# Autodesk Inventor assembly: SCHUNK- 1321170 Co-act EGP-C 40-N-N-KTOE, 0
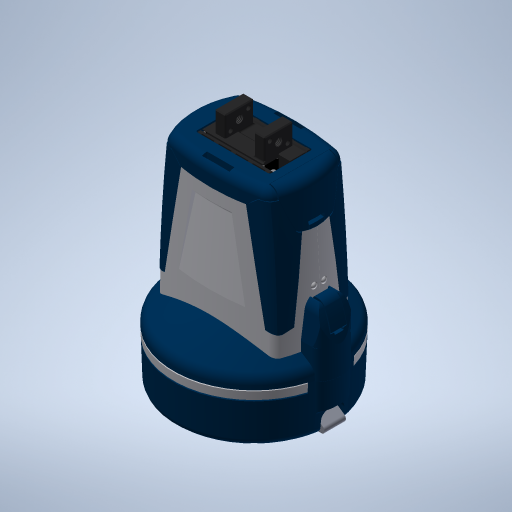
[picture p0: Inventor's stored thumbnail of the model, 512x512]
Saved by Autodesk Inventor 2023 (Build 270158000, 158)
## iProperties
Created: 2022-08-29
Part Number: SCHUNK- 1321170 Co-act EGP-C 40-N-N-KTOE, 0
Catalog Web Link: www.cadenas.de
Description: Co-act EGP-C-Collaborating gripper for small components
Vendor: SCHUNK
Document SubType Name: Assembly
Designer: psAdmin
Manufacturer: SCHUNK
Mass: 620 g
Surface Area: 1018.14 cm^2
Volume: 436.323 cm^3
Density: 1.42097 g/cm^3
Category: PARTsolutions
Company: SCHUNK
PSOL_IDENT_0: {$CADENAS_DATA/23d-libs/schunk/greifsysteme/greifmodule/co_act/co_act_egp_c/co_act_egp_c_asm_at.prj}
PSOL_IDENT_1: ,248 {VTYP=3D},{STYP=ASSTAB},{NB=SCHUNK- 1321170 Co-act EGP-C 40-N-N-KTOE, 0},{LINA=SCHUNK-1321170 C
PSOL_IDENT_2: o-act EGP-C 40-N-N-KTOE},{NN=Co-act EGP-C},{DATE=01.06.2022 15:24:31},{GEOMDATE=27.04.2022 08:42:34}
PSOL_IDENT_3: ,{VERSION=},{LINEID=20},{WBVAR=HUB},{WBNUMERIC=HUB}  {NB=SCHUNK- 1321170 Co-act EGP-C 40-N-N-KTOE, 0
PSOL_IDENT_4: },{LINA=SCHUNK-1321170 Co-act EGP-C 40-N-N-KTOE},{KT=DUMMY},{IDNR=1321170},{TYP=Co-act EGP-C 40-N-N-
PSOL_IDENT_5: KTOE},{ONLINE=Zur Produktseite},{INFOXX=https://schunk.com/gb_en/gripping-systems/product/63294-0},{
PSOL_IDENT_6: HUB=0},{CALC=../../../../produktbilder/icons/im0023672.png},{EPLAN=../../../../produktbilder/icons/i
PSOL_IDENT_7: m0021678.png},{HUBMAX=6.000},{PARTSERVER=1.000},{TYPBG=2.000},{TYP1=1.000},{TYPFLA=2.000},{WFLA=30.0
PSOL_IDENT_8: 00},{TYPEGP=EGP 40-N-N-B},{ROBOTER=KUKA LBR iiwa 7/14},{FLANSCH=Medien-Flansch Touch elektrisch},{LE
PSOL_IDENT_9: D=integriert},{FARBEN=Grün, Gelb, Rot},{SENSOREN=Ja, 2-fach induktiv},{HUBBACKE=6},{GREIFKRAFT=35/14
PSOL_IDENT_10: 0},{KRAFTPROBACKE=17.5/70},{WKSTGEWICHT=0.700},{FINGERLAENGE=50},{MASSEFINGER=0.080},{WIEDERHOLGENAU
PSOL_IDENT_11: I=0.020},{SCHLIESSOEFFNUN=0.2/0.2},{EIGENMASSE=0.620},{UMGEBUNGSTEMPER=5/55},{SCHUTZART=30},{KABELST
PSOL_IDENT_12: ECKEREND=M12},{KABELLAENGE=70},{NENNSPANN=24},{NENNSTROM=0.200},{MAXSTROM=2.000},{REGLERELEKTRONI=in
PSOL_IDENT_13: tegriert},{KOMMUNIKATIONSS=Digitale I/O},{ANZDIGITALEIO=4/2},{HOEHE=118.000},{HEGP=88.500},{CALCXX=h
PSOL_IDENT_14: ttps://schunk.com/de_de/services/digitale-services/berechnungs-und-auslegungstool-greifen/},{CALCXXX=
PSOL_IDENT_15: https://schunk.com/de_de/services/digitale-services/berechnungs-und-auslegungstool-greifen/},{EPLANX
PSOL_IDENT_16: X=https://eplandata.de/portal/portal.php?action=part-viewc&edpp=1.0&ev=1.9.11&lang=de_DE&clang=de_DE
PSOL_IDENT_17: &mf=SNK&lastmpg=.&mcat=_eplan&tab=c&mcatsel=SNK},{EPLANXXX=https://eplandata.de/portal/portal.php?ac
PSOL_IDENT_18: tion=part-viewc&edpp=1.0&ev=1.9.11&lang=de_DE&clang=de_DE&mf=SNK&lastmpg=.&mcat=_eplan&tab=c&mcatsel=
PSOL_IDENT_19: SNK},{CNSCTN=84798997},{EDZ=snk.1321170},{EPIMID=63294},{PPATH=co_act_egp_c_asmsbl.prj}
NB: SCHUNK- 1321170 Co-act EGP-C 40-N-N-KTOE, 0
NN: Co-act EGP-C
NT: Collaborating gripper for small components
NBSYN: SCHUNK- $IDNR. $TYP., $HUB.
LINA: SCHUNK-1321170 Co-act EGP-C 40-N-N-KTOE
CATALOG: SCHUNK
IDNR: 1321170
TYP: Co-act EGP-C 40-N-N-KTOE
ONLINE: To the product page
HUB: 0
CALC: ../../../../produktbilder/icons/im0023672.png
EPLAN: ../../../../produktbilder/icons/im0021678.png
ROBOTER: KUKA LBR iiwa 7/14
FLANSCH: Media flange touch electric
LED: integrated
FARBEN: green, yellow, red
SENSOREN: yes, inductive in two directions
HUBBACKE: 6
GREIFKRAFT: 35/140
KRAFTPROBACKE: 17.5/70
WKSTGEWICHT: 0.7
FINGERLAENGE: 50
MASSEFINGER: 0.08
WIEDERHOLGENAUI: 0.02
SCHLIESSOEFFNUN: 0.2/0.2
EIGENMASSE: 0.62
UMGEBUNGSTEMPER: 5/55
SCHUTZART: 30
KABELSTECKEREND: M12
KABELLAENGE: 70
NENNSPANN: 24
NENNSTROM: 0.2
MAXSTROM: 2
REGLERELEKTRONI: integrated
KOMMUNIKATIONSS: digital I/O
ANZDIGITALEIO: 4/2
CNSCTN: 84798997
SUPPLIER: SCHUNK
ARTICLENO: SCHUNK- 1321170 Co-act EGP-C 40-N-N-KTOE, 0
BOMINFO: SCHUNK-1321170 Co-act EGP-C 40-N-N-KTOE
CREATOR: CADENAS GmbH
Title: SCHUNK-1321170 Co-act EGP-C 40-N-N-KTOE
Author: Cadenas PARTsolutions
Comments: Collaborating gripper for small components
## Documents named in this file (4)
- C:\Users\Rober\Documents\Ingenieurinformatik\grop\catkin\src\grop\coactegpc\urdf\40\base\ktoe\SCHUNK- 1321170 Co-act EGP-C 40-N-N-KTOE, 0.iam
- C:\Users\Rober\Documents\Ingenieurinformatik\grop\catkin\src\grop\coactegpc\urdf\40\base\ktoe\ktoe.iam
- C:\Users\Rober\Documents\Ingenieurinformatik\grop\catkin\src\grop\coactegpc\urdf\40\base\ktoe\left.iam
- C:\Users\Rober\Documents\Ingenieurinformatik\grop\catkin\src\grop\coactegpc\urdf\40\base\ktoe\right.iam
## Components (3 placed, 3 different names)
1. ktoe:1 [sub-assembly]
2. left:1 [sub-assembly]
3. right:1 [sub-assembly]
## Relationships (4: Mate 3, Flush 1)
- [Flush]: ktoe:1 ↔ right:1
- [Mate]: ktoe:1 ↔ right:1
- [Mate]: ktoe:1 ↔ left:1
- [Mate]: ktoe:1 ↔ left:1
